# Autodesk Inventor assembly: ADF42030-Enclosure
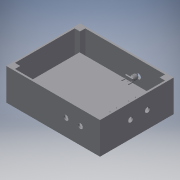
[picture p0: Inventor's stored thumbnail of the model, 180x180]
Saved by Autodesk Inventor 2018 (Build 220112000, 112)
## iProperties
Created: 2018-04-28
Part Number: ADF42030-Enclosure
Document SubType Name: Assembly
Designer: bbramman
Author: bbramman
## Documents named in this file (4)
- C:\Users\bbramman\OneDrive\Documents\Trapped Ion Research (Grad)\Electronics\pll-evalboard-synthesizer\Box CAD\ADF41020-Enclosure.iam
- C:\Users\bbramman\OneDrive\Documents\Trapped Ion Research (Grad)\Electronics\pll-evalboard-synthesizer\Box CAD\546-1590BBS-ADF41020.ipt
- C:\Users\bbramman\OneDrive\Documents\Trapped Ion Research (Grad)\Electronics\pll-evalboard-synthesizer\Box CAD\Power-Reg.iam
- C:\Users\bbramman\OneDrive\Documents\Trapped Ion Research (Grad)\Electronics\pll-evalboard-synthesizer\Box CAD\EV-ADF41020.iam
## Components (3 placed, 3 different names)
1. 546-1590BBS-ADF41020:1 — Insert:1, Mate:1
2. Power-Reg:1 [sub-assembly] — Insert:1
3. EV-ADF41020:1 [sub-assembly] — Mate:1
## Relationships (2: Insert 1, Mate 1)
- Insert:1 (-8.6106 mm): 546-1590BBS-ADF41020:1 ↔ Power-Reg:1
- Mate:1 (19.05 mm): 546-1590BBS-ADF41020:1 ↔ EV-ADF41020:1
